# Autodesk Inventor assembly: Koruza
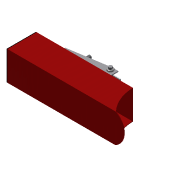
[picture p0: Inventor's stored thumbnail of the model, 180x180]
Saved by Autodesk Inventor 2015 (Build 190159000, 159)
## iProperties
Created: 2015-01-16
Part Number: Koruza
Document SubType Name: Assembly
Designer: Michal
Author: Michal
## Documents named in this file (12)
- C:\Users\Michal\Desktop\Michal\Prace\koruza\Koruza.iam
- C:\Users\Michal\Desktop\Michal\Prace\koruza\Case.ipt
- C:\Users\Michal\Desktop\Michal\Prace\koruza\U-profil 100x40 - pod case.ipt
- C:\Users\Michal\Desktop\Michal\Prace\koruza\L profil 100x100 základní.ipt
- C:\Users\Michal\Desktop\Michal\Prace\koruza\Šroub M12x160.ipt
- C:\Users\Michal\Desktop\Michal\Prace\koruza\ANSI B18.16.3M - Property Class 5 and 10 - Metric M12 x 1.75 Typ kovu.ipt
- C:\Users\Michal\Desktop\Michal\Prace\koruza\ISO 4035 - M12ISO.ipt
- C:\Users\Michal\Desktop\Michal\Prace\koruza\Šroub M12x70.ipt
- C:\Users\Michal\Desktop\Michal\Prace\koruza\Anténní držák.ipt
- C:\Users\Michal\Desktop\Michal\Prace\koruza\Šroub M4x10.ipt
- C:\Users\Michal\Desktop\Michal\Prace\koruza\ISO 4032 - M4ISO.ipt
- C:\Users\Michal\Desktop\Michal\Prace\koruza\Zadní kryt.ipt
## Components (14 placed, 11 different names)
1. Case:1 — Proti sobě:1, Stejný směr:1, Proti sobě:2, Proti sobě:13, Proti sobě:14, Proti sobě:15, Proti sobě:16, Proti sobě:17, Proti sobě:18, Proti sobě:25, Stejný směr:2, Stejný směr:3
2. U-profil 100x40 - pod case:1 — Proti sobě:1, Stejný směr:1, Proti sobě:2, Proti sobě:3, Proti sobě:4, Proti sobě:5, Proti sobě:10, Proti sobě:12, Proti sobě:20, Proti sobě:22
3. L profil 100x100 základní:1 — Proti sobě:3, Proti sobě:4, Proti sobě:6, Proti sobě:8, Proti sobě:23, Proti sobě:24
4. Šroub M12x160:1 — Proti sobě:5, Proti sobě:6, Proti sobě:7, Proti sobě:9, Proti sobě:11
5. ANSI B18.16.3M - Property Class 5 and 10 - Metric M12 x 1.75 Typ kovu:1 — Proti sobě:7, Proti sobě:8
6. ISO 4035 - M12ISO:1 — Proti sobě:9, Proti sobě:10
7. ISO 4035 - M12ISO:2 — Proti sobě:11, Proti sobě:12
8. Šroub M12x70:1 — Proti sobě:13, Proti sobě:14
9. Anténní držák:1 — Proti sobě:23, Proti sobě:24
10. Šroub M4x10:1 — Proti sobě:17, Proti sobě:18, Proti sobě:19
11. Šroub M4x10:2 — Proti sobě:15, Proti sobě:16, Proti sobě:21
12. ISO 4032 - M4ISO:1 — Proti sobě:21, Proti sobě:22
13. ISO 4032 - M4ISO:2 — Proti sobě:19, Proti sobě:20
14. Zadní kryt:1 — Proti sobě:25, Stejný směr:2, Stejný směr:3
## Relationships (28: Mate 25, Flush 3)
- Proti sobě:1 [Mate]: Case:1 ↔ U-profil 100x40 - pod case:1
- Stejný směr:1 [Flush]: Case:1 ↔ U-profil 100x40 - pod case:1
- Proti sobě:2 [Mate]: Case:1 ↔ U-profil 100x40 - pod case:1
- Proti sobě:3 [Mate] (25 mm): U-profil 100x40 - pod case:1 ↔ L profil 100x100 základní:1
- Proti sobě:4 [Mate]: U-profil 100x40 - pod case:1 ↔ L profil 100x100 základní:1
- Proti sobě:5 [Mate]: U-profil 100x40 - pod case:1 ↔ Šroub M12x160:1
- Proti sobě:6 [Mate]: L profil 100x100 základní:1 ↔ Šroub M12x160:1
- Proti sobě:7 [Mate]: Šroub M12x160:1 ↔ ANSI B18.16.3M - Property Class 5 and 10 - Metric M12 x 1.75 Typ kovu:1
- Proti sobě:8 [Mate]: L profil 100x100 základní:1 ↔ ANSI B18.16.3M - Property Class 5 and 10 - Metric M12 x 1.75 Typ kovu:1
- Proti sobě:9 [Mate]: Šroub M12x160:1 ↔ ISO 4035 - M12ISO:1
- Proti sobě:10 [Mate]: U-profil 100x40 - pod case:1 ↔ ISO 4035 - M12ISO:1
- Proti sobě:11 [Mate]: Šroub M12x160:1 ↔ ISO 4035 - M12ISO:2
- Proti sobě:12 [Mate]: U-profil 100x40 - pod case:1 ↔ ISO 4035 - M12ISO:2
- Proti sobě:13 [Mate]: Case:1 ↔ Šroub M12x70:1
- Proti sobě:14 [Mate]: Case:1 ↔ Šroub M12x70:1
- Proti sobě:15 [Mate]: Case:1 ↔ Šroub M4x10:2
- Proti sobě:16 [Mate]: Case:1 ↔ Šroub M4x10:2
- Proti sobě:17 [Mate]: Case:1 ↔ Šroub M4x10:1
- Proti sobě:18 [Mate]: Case:1 ↔ Šroub M4x10:1
- Proti sobě:19 [Mate]: Šroub M4x10:1 ↔ ISO 4032 - M4ISO:2
- Proti sobě:20 [Mate]: U-profil 100x40 - pod case:1 ↔ ISO 4032 - M4ISO:2
- Proti sobě:21 [Mate]: Šroub M4x10:2 ↔ ISO 4032 - M4ISO:1
- Proti sobě:22 [Mate]: U-profil 100x40 - pod case:1 ↔ ISO 4032 - M4ISO:1
- Proti sobě:23 [Mate]: L profil 100x100 základní:1 ↔ Anténní držák:1
- Proti sobě:24 [Mate]: L profil 100x100 základní:1 ↔ Anténní držák:1
- Proti sobě:25 [Mate]: Case:1 ↔ Zadní kryt:1
- Stejný směr:2 [Flush]: Case:1 ↔ Zadní kryt:1
- Stejný směr:3 [Flush]: Case:1 ↔ Zadní kryt:1
